# Autodesk Inventor assembly: EnsambleSuministroVapor
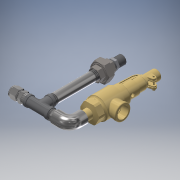
[picture p0: Inventor's stored thumbnail of the model, 180x180]
Saved by Autodesk Inventor 2017 (Build 210142000, 142)
## iProperties
Created: 2021-07-02
Part Number: EnsambleSuministroVapor
Document SubType Name: Assembly
Designer: USUARIO
Author: USUARIO
## Documents named in this file (8)
- D:\Laboratorio\Autoclave\Autoclave Horizontal\Con Precamara\2021\Autoclave 110L Biocacol OP2021110 #0045886XX\Modelo\Planos\EnsambleSuministroVapor.iam
- C:\Modelos 3D y DXF\Racores\B122 1-2x1-2.ipt
- C:\Modelos 3D y DXF\Racores\Universal1-2.ipt
- C:\Modelos 3D y DXF\Racores\Niple 1-2x5.ipt
- C:\Modelos 3D y DXF\Racores\User Library-Tee_Class300.ipt
- C:\Modelos 3D y DXF\Racores\CodoCalle.iam
- C:\Modelos 3D y DXF\Racores\User Library-Valvula-segur-popup-1-2.ipt
- C:\Modelos 3D y DXF\Racores\1-2-1-2-SwagelokCompany-3D-06-16-2021.ipt
## Components (7 placed, 7 different names)
1. B122 1-2x1-2:1
2. Universal1-2:1
3. Niple 1-2x5:1
4. User Library-Tee_Class300:1
5. CodoCalle:1 [sub-assembly]
6. User Library-Valvula-segur-popup-1-2:1
7. 1-2-1-2-SwagelokCompany-3D-06-16-2021:1
## Relationships (6: Insert 6)
- [Insert] (-12 mm): B122 1-2x1-2:1 ↔ Universal1-2:1
- [Insert] (-12 mm): Universal1-2:1 ↔ Niple 1-2x5:1
- [Insert] (12 mm): Niple 1-2x5:1 ↔ User Library-Tee_Class300:1
- [Insert] (-9 mm): CodoCalle:1 ↔ User Library-Valvula-segur-popup-1-2:1
- [Insert] (-12 mm): User Library-Tee_Class300:1 ↔ CodoCalle:1
- [Insert] (12 mm): User Library-Tee_Class300:1 ↔ 1-2-1-2-SwagelokCompany-3D-06-16-2021:1
## Named parameters: d78_d5 = -9 mm, d74_d32 = -12 mm
